# Autodesk Inventor assembly: TallBatteryBox
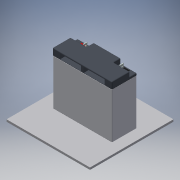
[picture p0: Inventor's stored thumbnail of the model, 180x180]
Saved by Autodesk Inventor 2016 (Build 200138000, 138)
## iProperties
Created: 2017-01-05
Part Number: TallBatteryBox
Document SubType Name: Assembly
Designer: james
Author: james
## Documents named in this file (3)
- C:\Users\james\Documents\Inventor\2017Ri3D\TallBatteryBox.iam
- C:\Users\james\Documents\Inventor\2017Ri3D\Floor.ipt
- C:\Users\james\Documents\Inventor\2017Ri3D\Battery.ipt
## Components (2 placed, 2 different names)
1. Floor:1 — Mate:1
2. Battery:1 — Mate:1
## Relationships (1: Mate 1)
- Mate:1: Floor:1 ↔ Battery:1
